# Autodesk Inventor assembly: RSX Assembly
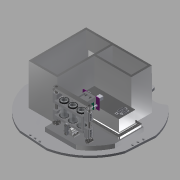
[picture p0: Inventor's stored thumbnail of the model, 180x180]
Saved by Autodesk Inventor 2017 (Build 210142000, 142)
## iProperties
Created: 2016-10-28
Part Number: RSX Assembly
Document SubType Name: Assembly
Designer: eschr_000
Author: eschr_000
## Documents named in this file (4)
- C:\Users\qupec\Desktop\UMD Near Space\STAR\CAD\Mechanical\CapTech\RSX Assembly.iam
- C:\Users\qupec\Desktop\UMD Near Space\STAR\CAD\Mechanical\CapTech\RSX Structure.ipt
- C:\Users\qupec\Desktop\UMD Near Space\STAR\CAD\Mechanical\CapTech\Keep Out RSX Deck.ipt
- C:\Users\qupec\Desktop\UMD Near Space\STAR\CAD\Mechanical\CapTech\RSX Deck.ipt
## Components (4 placed, 4 different names)
1. RSX Structure:1 — Mate:16, Mate:26, Mate:33, Mate:38, Mate:39, Mate:40
2. Keep Out RSX Deck:1 — Mate:16
3. RSX Deck:1 — Mate:26, Mate:33, Mate:38, Mate:41
4. Full payload assembly mk 2:1 [sub-assembly] — Mate:39, Mate:40, Mate:41
## Relationships (7: Mate 7)
- Mate:16: RSX Structure:1 ↔ Keep Out RSX Deck:1
- Mate:26: RSX Structure:1 ↔ RSX Deck:1
- Mate:33: RSX Structure:1 ↔ RSX Deck:1
- Mate:38: RSX Structure:1 ↔ RSX Deck:1
- Mate:39: RSX Structure:1 ↔ Full payload assembly mk 2:1
- Mate:40: RSX Structure:1 ↔ Full payload assembly mk 2:1
- Mate:41: RSX Deck:1 ↔ Full payload assembly mk 2:1
